# Autodesk Inventor assembly: Bil
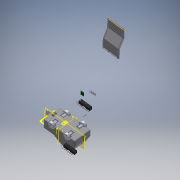
[picture p0: Inventor's stored thumbnail of the model, 180x180]
Saved by Autodesk Inventor 2019 (Build 230136000, 136)
## iProperties
Created: 2018-12-03
Part Number: Bil
Document SubType Name: Assembly
Designer: Filip
Author: Filip
## Documents named in this file (15)
- C:\Users\Filip\Desktop\CAD\Bil\Delar\Bil.iam
- C:\Users\Filip\Desktop\CAD\Bil\Delar\18650 Battery Holder.ipt
- C:\Users\Filip\Desktop\CAD\Bil\Delar\Samsung INR18650-29R.ipt
- C:\Users\Filip\Desktop\CAD\Bil\Delar\Solderless Breadboard.ipt
- C:\Users\Filip\Desktop\CAD\Bil\Delar\Hjul.ipt
- C:\Users\Filip\Desktop\CAD\Bil\Delar\battery_controller.iam
- C:\Users\Filip\Desktop\CAD\Bil\Delar\RapberryPiZero.ipt
- C:\Users\Filip\Desktop\CAD\Bil\Delar\type_fa130.iam
- C:\Users\Filip\Desktop\CAD\Bil\Delar\Bas.ipt
- C:\Users\Filip\Desktop\CAD\Bil\Delar\knapp.ipt
- C:\Users\Filip\Desktop\CAD\Bil\Delar\L298N.ipt
- C:\Users\Filip\Desktop\CAD\Bil\Delar\L298N_CPY.ipt
- C:\Users\Filip\Desktop\CAD\Bil\Delar\Stiftlist.ipt
- C:\Users\Filip\Desktop\CAD\Bil\Delar\Lock.ipt
- C:\Users\Filip\Downloads\raspberry-pi-camera-module-v2-1.snapshot.3\RspCameraMia.iam
## Components (22 placed, 14 different names)
1. RapberryPiZero:1 — Mate:27
2. 18650 Battery Holder:1 — Rigid:1, Mate:30
3. 18650 Battery Holder:2 — Rigid:2, Mate:29
4. Samsung INR18650-29R:1 — Rigid:2
5. Samsung INR18650-29R:2 — Rigid:1
6. Solderless Breadboard:1 — Mate:28
7. Hjul:1 — Insert:4
8. Hjul:2 — Insert:5
9. Hjul:3 — Insert:3
10. Hjul:4 — Insert:2
11. battery_controller:1 [sub-assembly] — Mate:31
12. motor:1 [sub-assembly] — Insert:4, Mate:22
13. motor:2 [sub-assembly] — Insert:5, Mate:23
14. motor:3 [sub-assembly] — Insert:2, Mate:20
15. motor:4 [sub-assembly] — Insert:3, Mate:21
16. Bas:1 — Mate:6, Mate:7, Flush:1, Mate:20, Mate:21, Mate:22, Mate:23, Mate:27, Mate:28, Mate:29, Mate:30, Mate:31
17. knapp:1
18. L298N:1 — Mate:6
19. L298N_CPY:1 — Mate:7
20. Stiftlist:1
21. Lock:1 — Flush:1
22. RspCameraMia:1 [sub-assembly]
## Relationships (18: Mate 11, Insert 4, WeldJoint 2, Flush 1)
- Insert:2 (7.62 mm): Hjul:4 ↔ motor:3
- Insert:3 (7.62 mm): Hjul:3 ↔ motor:4
- Insert:4 (7.62 mm): Hjul:1 ↔ motor:1
- Insert:5 (7.62 mm): Hjul:2 ↔ motor:2
- Rigid:1 [WeldJoint]: 18650 Battery Holder:1 ↔ Samsung INR18650-29R:2
- Rigid:2 [WeldJoint]: 18650 Battery Holder:2 ↔ Samsung INR18650-29R:1
- Mate:6: Bas:1 ↔ L298N:1
- Mate:7: Bas:1 ↔ L298N_CPY:1
- Flush:1: Bas:1 ↔ Lock:1
- Mate:20: motor:3 ↔ Bas:1
- Mate:21: motor:4 ↔ Bas:1
- Mate:22: motor:1 ↔ Bas:1
- Mate:23: motor:2 ↔ Bas:1
- Mate:27: RapberryPiZero:1 ↔ Bas:1
- Mate:28: Solderless Breadboard:1 ↔ Bas:1
- Mate:29: 18650 Battery Holder:2 ↔ Bas:1
- Mate:30: 18650 Battery Holder:1 ↔ Bas:1
- Mate:31: battery_controller:1 ↔ Bas:1
